# Autodesk Inventor assembly: Arm Yay
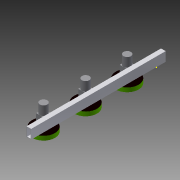
[picture p0: Inventor's stored thumbnail of the model, 180x180]
Saved by Autodesk Inventor 2015 (Build 190159000, 159)
## iProperties
Created: 2015-01-11
Part Number: Arm Yay
Document SubType Name: Assembly
Designer: chapale16
Author: chapale16
## Documents named in this file (4)
- \\lhssvr02\Homedirs\Robotics Club\CAD Model 2015\Game Components\The Tote Collector-Arms\Tote Collector Arm.iam
- \\lhssvr02\Homedirs\Robotics Club\CAD Model 2015\Game Components\The Tote Collector-Arms\P60 Gear Box.ipt
- \\lhssvr02\Homedirs\Robotics Club\CAD Model 2015\Game Components\The Tote Collector-Arms\Arm.ipt
- \\lhssvr02\Homedirs\Robotics Club\CAD Model 2015\Game Components\The Tote Collector-Arms\collector arm wheel.ipt
## Components (7 placed, 3 different names)
1. P60 Gear Box:1 — Mate:3, Mate:4, Flush:1, Flush:5
2. P60 Gear Box:2 — Mate:2, Mate:5, Flush:2, Flush:6
3. P60 Gear Box:3 — Mate:1, Mate:6, Flush:3, Flush:4
4. Arm:1 — Mate:1, Mate:2, Mate:3, Flush:4, Flush:5, Flush:6
5. collector arm wheel:1 — Mate:6, Flush:3
6. collector arm wheel:2 — Mate:5, Flush:2
7. collector arm wheel:3 — Mate:4, Flush:1
## Relationships (12: Mate 6, Flush 6)
- Mate:1: P60 Gear Box:3 ↔ Arm:1
- Mate:2: P60 Gear Box:2 ↔ Arm:1
- Mate:3: P60 Gear Box:1 ↔ Arm:1
- Mate:4: P60 Gear Box:1 ↔ collector arm wheel:3
- Mate:5: P60 Gear Box:2 ↔ collector arm wheel:2
- Mate:6: P60 Gear Box:3 ↔ collector arm wheel:1
- Flush:1: P60 Gear Box:1 ↔ collector arm wheel:3
- Flush:2: P60 Gear Box:2 ↔ collector arm wheel:2
- Flush:3: P60 Gear Box:3 ↔ collector arm wheel:1
- Flush:4: P60 Gear Box:3 ↔ Arm:1
- Flush:5: P60 Gear Box:1 ↔ Arm:1
- Flush:6: P60 Gear Box:2 ↔ Arm:1
